# Autodesk Inventor assembly: OringFixture
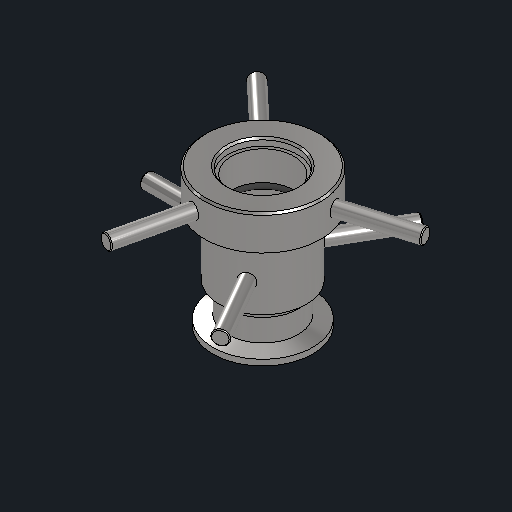
[picture p0: Inventor's stored thumbnail of the model, 512x512]
Saved by Autodesk Inventor 2026 (Build 300175050, 175E)
## iProperties
Created: 2022-12-02
Part Number: OringFixture
Document SubType Name: Assembly
Designer: kuzmin
Author: kuzmin
## Documents named in this file (6)
- C:\Users\queez\Dropbox\Drawings\PIHTI\PALP\OringFixture.iam
- C:\Users\queez\Dropbox\Drawings\PIHTI\PALP\Oring-seal\Oring_KF_part.iam
- C:\Users\queez\Dropbox\Drawings\PIHTI\PALP\Oring-seal\OringPressingRing.ipt
- C:\Users\queez\Dropbox\Drawings\PIHTI\PALP\Oring-seal\Oring.ipt
- C:\Users\queez\Dropbox\Drawings\PIHTI\PALP\Oring-seal\Oring_M48-2_nut.ipt
- C:\Users\queez\Dropbox\Drawings\PIHTI\PALP\Oring-seal\OringM5Wrench.ipt
## Components (10 placed, 5 different names)
1. Oring_KF_part:1 [sub-assembly] — Mate:1, Mate:2, Mate:3, Mate:4, Tangent:1, Mate:5, Rigid:1, Rigid:2, Rigid:3
2. OringPressingRing:1 — Mate:5, Tangent:2, Rotational:1
3. Oring:1 — Mate:4, Tangent:1, Tangent:2
4. Oring_M48-2_nut:1 — Rotational:1, Rotational:2, Rotational:3, Rotational:4
5. OringM5Wrench:1 — Rotational:2
6. OringM5Wrench:2 — Rotational:4
7. OringM5Wrench:3 — Rotational:3
8. OringM5Wrench:4 — Rigid:1
9. OringM5Wrench:5 — Rigid:2
10. OringM5Wrench:6 — Rigid:3
## Relationships (14: Mate 5, RevoluteJoint 4, WeldJoint 3, Tangent 2)
- Mate:1: Oring_KF_part:1
- Mate:2: Oring_KF_part:1
- Mate:3: Oring_KF_part:1
- Mate:4: Oring_KF_part:1 ↔ Oring:1
- Tangent:1: Oring_KF_part:1 ↔ Oring:1
- Mate:5: Oring_KF_part:1 ↔ OringPressingRing:1
- Tangent:2: OringPressingRing:1 ↔ Oring:1
- Rotational:1 [RevoluteJoint]: OringPressingRing:1 ↔ Oring_M48-2_nut:1
- Rotational:2 [RevoluteJoint]: Oring_M48-2_nut:1 ↔ OringM5Wrench:1
- Rotational:3 [RevoluteJoint]: Oring_M48-2_nut:1 ↔ OringM5Wrench:3
- Rotational:4 [RevoluteJoint]: Oring_M48-2_nut:1 ↔ OringM5Wrench:2
- Rigid:1 [WeldJoint]: Oring_KF_part:1 ↔ OringM5Wrench:4
- Rigid:2 [WeldJoint]: Oring_KF_part:1 ↔ OringM5Wrench:5
- Rigid:3 [WeldJoint]: Oring_KF_part:1 ↔ OringM5Wrench:6
